# Autodesk Inventor assembly: 左後脚ユニット1_MIR
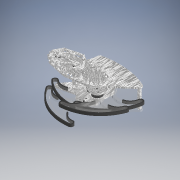
[picture p0: Inventor's stored thumbnail of the model, 180x180]
Saved by Autodesk Inventor 2020 (Build 240168000, 168)
## iProperties
Created: 2019-07-24
Part Number: 左後脚ユニット1_MIR
Document SubType Name: Assembly
Designer: 雪村
Mass: 208.087 g
Surface Area: 1099.86 cm^2
Volume: 100.406 cm^3
Density: 2.07245 g/cm^3
Author: 雪村
## Documents named in this file (12)
- C:\Users\white\Documents\SRDC\SRDC\Inventor_2017\2018年機体\2020年4年機体\右後脚ユニット1.iam
- C:\Users\white\Documents\SRDC\SRDC\Inventor_2017\2018年機体\2020年4年機体\後脚内フレーム1_MIR.ipt
- C:\Users\white\Documents\SRDC\SRDC\Inventor_2017\2018年機体\2020年4年機体\脚クランク1.iam
- C:\Users\white\Documents\SRDC\SRDC\Inventor_2017\2018年機体\パーツ\オイレスフランジ付き12142006.ipt
- C:\Users\white\Documents\SRDC\SRDC\Inventor_2017\2018年機体\2020年4年機体\後脚ギアトレイン1_MIR.iam
- C:\Users\white\Documents\SRDC\SRDC\Inventor_2017\2018年機体\パーツ\オイレスフランジ付き14162202.5.ipt
- C:\Users\white\Documents\SRDC\SRDC\Inventor_2017\2018年機体\2020年4年機体\脚最終段カム1.ipt
- C:\Users\white\Documents\SRDC\SRDC\Inventor_2017\2018年機体\2020年4年機体\歯車m2.z14.ipt
- C:\Users\white\Documents\SRDC\SRDC\Inventor_2017\2018年機体\2020年4年機体\後脚ユニット締結パーツ1_MIR.ipt
- C:\Users\white\Documents\SRDC\SRDC\Inventor_2017\2018年機体\2020年4年機体\前脚外フレーム1_MIR_MIR.ipt
- C:\Users\white\Documents\SRDC\SRDC\Inventor_2017\2018年機体\パーツ\スペーサーm3,35.ipt
- C:\Users\white\Documents\SRDC\SRDC\Inventor_2017\2018年機体\2020年4年機体\ヘッケン＋揺動節1_MIR.iam
## Components (16 placed, 11 different names)
1. 後脚内フレーム1_MIR:1 — 挿入:1, 挿入:6, 挿入:9, 挿入:10, 挿入:11
2. 脚クランク1:1 [sub-assembly] — 挿入:2, 挿入:3, 挿入:16, 挿入:17, 挿入:18, 挿入:19
3. オイレスフランジ付き12142006:1 — 挿入:1, 挿入:8
4. 後脚ギアトレイン1_MIR:1 [sub-assembly] — 挿入:7, メイト:5
5. オイレスフランジ付き14162202.5:1 — 挿入:6, 挿入:7
6. 脚最終段カム1:1 — 挿入:2, 挿入:3, 挿入:4, 挿入:5, 挿入:8
7. 歯車m2.z14:1 — 挿入:4, 挿入:5
8. 後脚ユニット締結パーツ1_MIR:1 — 挿入:14, 挿入:15, メイト:5
9. 前脚外フレーム1_MIR_MIR:1 — 挿入:12, 挿入:13, 挿入:14, 挿入:15
10. スペーサーm3,35:1 — 挿入:10, メイト:1, メイト:2, メイト:3, メイト:4
11. スペーサーm3,35:2 — 挿入:9, 挿入:13
12. スペーサーm3,35:3 — 挿入:11, 挿入:12
13. ヘッケン＋揺動節1_MIR:1 [sub-assembly] — 挿入:16, メイト:3
14. ヘッケン＋揺動節1_MIR:2 [sub-assembly] — 挿入:17, メイト:1
15. ヘッケン＋揺動節1_MIR:3 [sub-assembly] — 挿入:18, メイト:4
16. ヘッケン＋揺動節1_MIR:4 [sub-assembly] — 挿入:19, メイト:2
## Relationships (24: Insert 19, Mate 5)
- 挿入:1 [Insert]: 後脚内フレーム1_MIR:1 ↔ オイレスフランジ付き12142006:1
- 挿入:2 [Insert]: 脚クランク1:1 ↔ 脚最終段カム1:1
- 挿入:3 [Insert]: 脚クランク1:1 ↔ 脚最終段カム1:1
- 挿入:4 [Insert]: 脚最終段カム1:1 ↔ 歯車m2.z14:1
- 挿入:5 [Insert]: 脚最終段カム1:1 ↔ 歯車m2.z14:1
- 挿入:6 [Insert]: 後脚内フレーム1_MIR:1 ↔ オイレスフランジ付き14162202.5:1
- 挿入:7 [Insert]: 後脚ギアトレイン1_MIR:1 ↔ オイレスフランジ付き14162202.5:1
- 挿入:8 [Insert]: オイレスフランジ付き12142006:1 ↔ 脚最終段カム1:1
- 挿入:9 [Insert]: 後脚内フレーム1_MIR:1 ↔ スペーサーm3,35:2
- 挿入:10 [Insert]: 後脚内フレーム1_MIR:1 ↔ スペーサーm3,35:1
- 挿入:11 [Insert]: 後脚内フレーム1_MIR:1 ↔ スペーサーm3,35:3
- 挿入:12 [Insert]: 前脚外フレーム1_MIR_MIR:1 ↔ スペーサーm3,35:3
- 挿入:13 [Insert]: 前脚外フレーム1_MIR_MIR:1 ↔ スペーサーm3,35:2
- 挿入:14 [Insert]: 後脚ユニット締結パーツ1_MIR:1 ↔ 前脚外フレーム1_MIR_MIR:1
- 挿入:15 [Insert]: 後脚ユニット締結パーツ1_MIR:1 ↔ 前脚外フレーム1_MIR_MIR:1
- 挿入:16 [Insert]: 脚クランク1:1 ↔ ヘッケン＋揺動節1_MIR:1
- 挿入:17 [Insert]: 脚クランク1:1 ↔ ヘッケン＋揺動節1_MIR:2
- 挿入:18 [Insert]: 脚クランク1:1 ↔ ヘッケン＋揺動節1_MIR:3
- 挿入:19 [Insert]: 脚クランク1:1 ↔ ヘッケン＋揺動節1_MIR:4
- メイト:1 [Mate]: スペーサーm3,35:1 ↔ ヘッケン＋揺動節1_MIR:2
- メイト:2 [Mate]: スペーサーm3,35:1 ↔ ヘッケン＋揺動節1_MIR:4
- メイト:3 [Mate]: スペーサーm3,35:1 ↔ ヘッケン＋揺動節1_MIR:1
- メイト:4 [Mate]: スペーサーm3,35:1 ↔ ヘッケン＋揺動節1_MIR:3
- メイト:5 [Mate]: 後脚ギアトレイン1_MIR:1 ↔ 後脚ユニット締結パーツ1_MIR:1
